# Autodesk Inventor assembly: ASY ДМФ 030 кольцо со шпильками корма
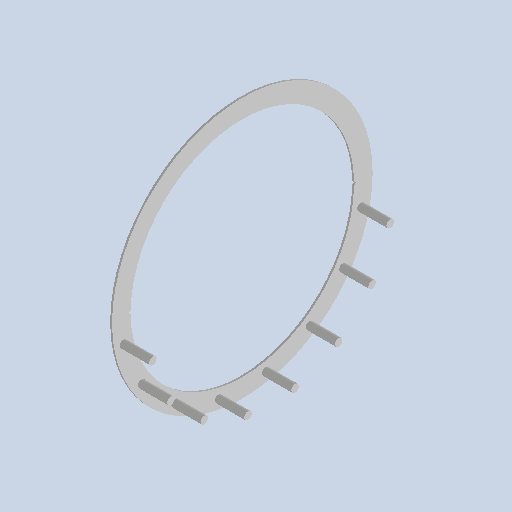
[picture p0: Inventor's stored thumbnail of the model, 512x512]
Saved by Autodesk Inventor 2024.2 (Build 282272000, 272)
## iProperties
Created: 2024-04-23
Part Number: ASY ДМФ 030 кольцо со шпильками корма
Document SubType Name: Assembly
Designer: admin
Author: admin
## Documents named in this file (4)
- C:\Users\user\YandexDisk\домашниий пк\Inventor\DMF-Disk-Micro-Filter\ASY ДМФ 030 кольцо со шпильками корма.iam
- C:\Users\user\YandexDisk\домашниий пк\Inventor\DMF-Disk-Micro-Filter\ДМФ 031 кольцо под шпильки НОС.ipt
- C:\Users\user\YandexDisk\домашниий пк\Inventor\DMF-Disk-Micro-Filter\ДМФ 000 размеры.ipt
- C:\Users\user\YandexDisk\домашниий пк\Inventor\DMF-Disk-Micro-Filter\ДМС 033 шпилька 3.ipt
## Components (9 placed, 2 different names)
1. ДМС 010 кольцо под шпильки:1 — Mate:1, Rigid:1
2. ДМС 033 шпилька 3:1 — Rigid:1
3. ДМС 033 шпилька 3:2
4. ДМС 033 шпилька 3:3
5. ДМС 033 шпилька 3:4
6. ДМС 033 шпилька 3:5
7. ДМС 033 шпилька 3:6
8. ДМС 033 шпилька 3:7
9. ДМС 033 шпилька 3:8
## Component patterns: (8 elements, first: ДМС 033 шпилька 3:1)
## Relationships (2: Mate 1, WeldJoint 1)
- Mate:1: ДМС 010 кольцо под шпильки:1
- Rigid:1 [WeldJoint]: ДМС 010 кольцо под шпильки:1 ↔ ДМС 033 шпилька 3:1
